# Autodesk Inventor assembly: Chest
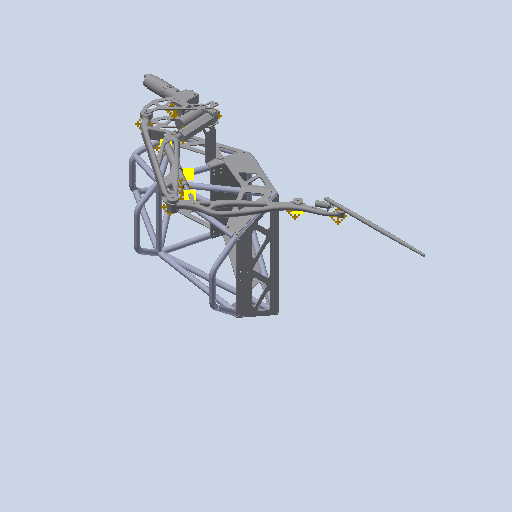
[picture p0: Inventor's stored thumbnail of the model, 512x512]
Saved by Autodesk Inventor 2025.2 (Build 292293000, 293)
## iProperties
Created: 2025-02-15
Part Number: Chest
Document SubType Name: Assembly
Designer: valer
Author: valer
## Documents named in this file (8)
- D:\str1ker\cad\Chest.iam
- D:\str1ker\cad\ChestWireframe.ipt
- D:\str1ker\cad\ChestFront.ipt
- D:\str1ker\cad\ChestSide.ipt
- D:\str1ker\cad\ChestSideMirror.ipt
- D:\str1ker\cad\ArmWithBase.iam
- D:\str1ker\cad\ChestMiddle.ipt
- D:\str1ker\cad\Chest.ipt
## Components (7 placed, 7 different names)
1. ChestWireframe:1 — Flush:1, Flush:2, Mate:1, Flush:3, Mate:2, Mate:3, Mate:4, Mate:7, Mate:8, Mate:9, Mate:10, Mate:11, Mate:12, Mate:13, Mate:14, Flush:5, Mate:16, Mate:17
2. ChestFront:1 — Mate:2, Mate:3, Mate:4
3. ChestSide:1 — Mate:7, Mate:8, Mate:9, Mate:10, Mate:11
4. ChestSideMirror:1 — Mate:12, Mate:13, Mate:14
5. ArmWithBase:1 [sub-assembly] — Mate:15, Flush:6
6. ChestMiddle:1 — Flush:5, Mate:15, Flush:6
7. Chest:1 — Mate:16, Mate:17
## Relationships (20: Mate 15, Flush 5)
- Flush:1: ChestWireframe:1
- Flush:2: ChestWireframe:1
- Mate:1: ChestWireframe:1
- Flush:3: ChestWireframe:1
- Mate:2: ChestWireframe:1 ↔ ChestFront:1
- Mate:3: ChestWireframe:1 ↔ ChestFront:1
- Mate:4 (9.525 mm): ChestWireframe:1 ↔ ChestFront:1
- Mate:7 (11.1125 mm): ChestWireframe:1 ↔ ChestSide:1
- Mate:8: ChestWireframe:1 ↔ ChestSide:1
- Mate:9: ChestWireframe:1 ↔ ChestSide:1
- Mate:10: ChestWireframe:1 ↔ ChestSide:1
- Mate:11: ChestWireframe:1 ↔ ChestSide:1
- Mate:12 (11.1125 mm): ChestWireframe:1 ↔ ChestSideMirror:1
- Mate:13: ChestWireframe:1 ↔ ChestSideMirror:1
- Mate:14: ChestWireframe:1 ↔ ChestSideMirror:1
- Flush:5 (-9.525 mm): ChestWireframe:1 ↔ ChestMiddle:1
- Mate:15: ArmWithBase:1 ↔ ChestMiddle:1
- Flush:6: ArmWithBase:1 ↔ ChestMiddle:1
- Mate:16: ChestWireframe:1 ↔ Chest:1
- Mate:17: ChestWireframe:1 ↔ Chest:1
